# Autodesk Inventor assembly: Assemblage absorbeur
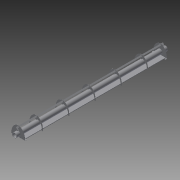
[picture p0: Inventor's stored thumbnail of the model, 180x180]
Saved by Autodesk Inventor 2015 SP1 (Build 190203100, 203)
## iProperties
Created: 2015-05-01
Part Number: Assemblage absorbeur
Document SubType Name: Assembly
Designer: Cyril
Author: Cyril
## Documents named in this file (7)
- C:\Users\Cyril\Documents\OSE FR\Concentrateur solaire\Absorbeur\Assemblage absorbeur E-O.iam
- C:\Users\Cyril\Documents\OSE FR\Concentrateur solaire\Absorbeur\Poutre centrale.ipt
- C:\Users\Cyril\Documents\OSE FR\Concentrateur solaire\Absorbeur\Patron.ipt
- C:\Users\Cyril\Documents\OSE FR\Concentrateur solaire\Absorbeur\Bouchon.ipt
- C:\Users\Cyril\Documents\OSE FR\Concentrateur solaire\Absorbeur\Raccord.ipt
- C:\Users\Cyril\Documents\OSE FR\Concentrateur solaire\Absorbeur\Vitre.ipt
- C:\Users\Cyril\Documents\OSE FR\Concentrateur solaire\Absorbeur\Tube.ipt
## Components (12 placed, 6 different names)
1. Poutre centrale:1 — Mate:1, Mate:2, Mate:3, Mate:4, Mate:9, Mate:10, Angle:1, Mate:15, Mate:16, Mate:17, Mate:18, Mate:25, Mate:26, Mate:29, Mate:30
2. Bouchon:1 — Mate:29, Mate:30, Mate:31, Mate:33
3. Bouchon:2 — Mate:25, Mate:26, Mate:32
4. Raccord:1 — Mate:9, Mate:10, Mate:18
5. Raccord:2 — Mate:15, Mate:16, Mate:17
6. Vitre:1 — Mate:27, Mate:28, Mate:31, Mate:32
7. Tube:1 — Mate:33
8. Patron:1 — Mate:3, Mate:4
9. Patron:2
10. Patron:3
11. Patron:4
12. Patron:5 — Mate:28
## Component patterns: (5 elements, first: Patron:1)
## Relationships (20: Mate 19, Angle 1)
- Mate:1: Poutre centrale:1
- Mate:2: Poutre centrale:1
- Mate:3: Poutre centrale:1 ↔ Patron:1
- Mate:4: Poutre centrale:1 ↔ Patron:1
- Mate:9: Poutre centrale:1 ↔ Raccord:1
- Mate:10: Poutre centrale:1 ↔ Raccord:1
- Angle:1 (45 deg): Poutre centrale:1
- Mate:15: Poutre centrale:1 ↔ Raccord:2
- Mate:16: Poutre centrale:1 ↔ Raccord:2
- Mate:17: Poutre centrale:1 ↔ Raccord:2
- Mate:18: Poutre centrale:1 ↔ Raccord:1
- Mate:25: Poutre centrale:1 ↔ Bouchon:2
- Mate:26: Poutre centrale:1 ↔ Bouchon:2
- Mate:27: Vitre:1
- Mate:28: Vitre:1 ↔ Patron:5
- Mate:29: Poutre centrale:1 ↔ Bouchon:1
- Mate:30: Poutre centrale:1 ↔ Bouchon:1
- Mate:31 (5 mm): Bouchon:1 ↔ Vitre:1
- Mate:32 (5 mm): Bouchon:2 ↔ Vitre:1
- Mate:33: Bouchon:1 ↔ Tube:1
